# Autodesk Inventor assembly: SAFRS-A-0002
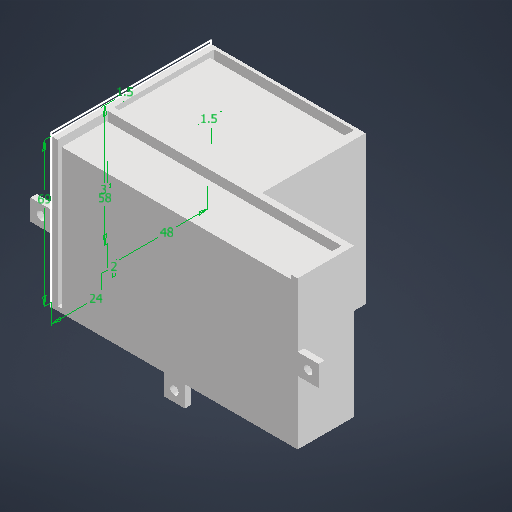
[picture p0: Inventor's stored thumbnail of the model, 512x512]
Saved by Autodesk Inventor 2026.2 (Build 302298000, 298)
## iProperties
Created: 2025-11-26
Part Number: SAFRS-A-0002
Document SubType Name: Assembly
Designer: jaewook
Author: jaewook
Title: Battery Pack Assembly
## Documents named in this file (4)
- C:\Users\jk000\OneDrive\Desktop\git\SAFRS\mechanical\inventor\02__subassemblies\battery_pack.iam
- C:\Users\jk000\OneDrive\Desktop\git\SAFRS\mechanical\inventor\01_parts\battery_pack_1.ipt
- C:\Users\jk000\OneDrive\Desktop\git\SAFRS\mechanical\inventor\01_parts\battery_pack_2.ipt
- C:\Users\jk000\OneDrive\Desktop\git\SAFRS\mechanical\inventor\01_parts\battery_base.ipt
## Components (3 placed, 3 different names)
1. battery_pack_1:1 — 강체:1
2. battery_pack_2:1 — 강체:2
3. battery_base:1 — 강체:1, 강체:2
## Relationships (2: WeldJoint 2)
- 강체:1 [WeldJoint]: battery_pack_1:1 ↔ battery_base:1
- 강체:2 [WeldJoint]: battery_pack_2:1 ↔ battery_base:1
